# Autodesk Inventor assembly: Stage2
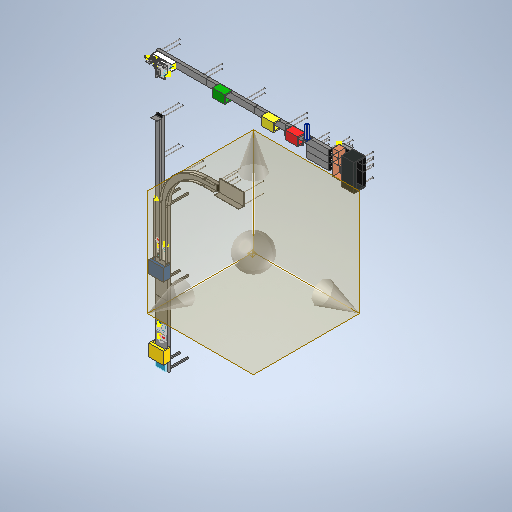
[picture p0: Inventor's stored thumbnail of the model, 512x512]
Saved by Autodesk Inventor 2025.1 (Build 291241000, 241)
## iProperties
Created: 2025-02-26
Part Number: Stage2
Document SubType Name: Assembly
Designer: yovan
Author: yovan
## Documents named in this file (27)
- C:\Users\yovan\Desktop\APM\ausol-apm.github.io\project\Design and simulation\Inventor\NXModeling\Stage2.iam
- C:\Users\yovan\Desktop\APM\ausol-apm.github.io\project\Design and simulation\Inventor\NXModeling\Assembler.ipt
- C:\Users\yovan\Desktop\APM\ausol-apm.github.io\project\Design and simulation\Inventor\NXModeling\ConveyorsStage2-3.ipt
- C:\Users\yovan\Desktop\APM\ausol-apm.github.io\project\Design and simulation\Inventor\Modelado juguetes\Barco\BarcoFinal.iam
- C:\Users\yovan\Desktop\APM\ausol-apm.github.io\project\Design and simulation\Inventor\Modelado juguetes\Barco\Piezabarcosuperior.ipt
- C:\Users\yovan\Desktop\APM\ausol-apm.github.io\project\Design and simulation\Inventor\Modelado juguetes\Barco\Timon.ipt
- C:\Users\yovan\Desktop\APM\ausol-apm.github.io\project\Design and simulation\Inventor\Modelado juguetes\Barco\PiezaTimon.ipt
- C:\Users\yovan\Desktop\APM\ausol-apm.github.io\project\Design and simulation\Inventor\Modelado juguetes\Moto\EnsamblajeMoto.iam
- C:\Users\yovan\Desktop\APM\ausol-apm.github.io\project\Design and simulation\Inventor\Modelado juguetes\Moto\Llanta.ipt
- C:\Users\yovan\Desktop\APM\ausol-apm.github.io\project\Design and simulation\Inventor\NXModeling\Sensor.ipt
- C:\Users\yovan\Desktop\APM\ausol-apm.github.io\project\Design and simulation\Inventor\Modelado juguetes\Casa\TechoCasa.ipt
- C:\Users\yovan\Desktop\APM\ausol-apm.github.io\project\Design and simulation\Inventor\Modelado juguetes\Casa\EnsamblajeCasa.iam
- C:\Users\yovan\Desktop\APM\ausol-apm.github.io\project\Design and simulation\Inventor\NXModeling\PneumaticActuator\PneummaticActuator.iam
- C:\Users\yovan\Desktop\APM\ausol-apm.github.io\project\Design and simulation\Inventor\NXModeling\Caja grande.ipt
- C:\Users\yovan\Desktop\APM\ausol-apm.github.io\project\Design and simulation\Inventor\NXModeling\Caja pequeña.ipt
- C:\Users\yovan\Desktop\APM\ausol-apm.github.io\project\Design and simulation\Inventor\NXModeling\ConveyorS&F.ipt
- C:\Users\yovan\Desktop\APM\ausol-apm.github.io\project\Design and simulation\Inventor\NXModeling\BiggerPneumatic\biggerAct.iam
- C:\Users\yovan\Desktop\APM\ausol-apm.github.io\project\Design and simulation\Inventor\NXModeling\Camera.ipt
- C:\Users\yovan\Desktop\APM\ausol-apm.github.io\project\Design and simulation\Inventor\NXModeling\smallerActuator\PneummaticActuatorSmall.iam
- C:\Users\yovan\Desktop\APM\ausol-apm.github.io\project\Design and simulation\Inventor\InjectionSetUp_RoboticCell\OutMold.ipt
- C:\Users\yovan\Desktop\APM\ausol-apm.github.io\project\Design and simulation\Inventor\Modelado juguetes\Casa\ParedDelanteraCasa.ipt
- C:\Users\yovan\Desktop\APM\ausol-apm.github.io\project\Design and simulation\Inventor\Modelado juguetes\Casa\ParedLateralCasa.ipt
- C:\Users\yovan\Desktop\APM\ausol-apm.github.io\project\Design and simulation\Inventor\Modelado juguetes\Casa\ParedTraseraCasa.ipt
- C:\Users\yovan\Desktop\APM\ausol-apm.github.io\project\Design and simulation\Inventor\Modelado juguetes\Casa\Puerta.ipt
- C:\Users\yovan\Desktop\APM\ausol-apm.github.io\project\Design and simulation\Inventor\Modelado juguetes\Casa\EnsamblajeCasaFinal.iam
- C:\Users\yovan\Desktop\APM\ausol-apm.github.io\project\Design and simulation\Inventor\Modelado juguetes\Moto\EnsamblajeMotoFinal.iam
- C:\Users\yovan\Desktop\APM\ausol-apm.github.io\project\Design and simulation\Inventor\Modelado juguetes\Barco\Inferior.ipt
## Components (71 placed, 26 different names)
1. Assembler:1 — Flush:1, Mate:1, Mate:3, Mate:4, Mate:8, Mate:9, Mate:10, Insert:4, Insert:5, Insert:6, Mate:11, Mate:12, Insert:7, Mate:13, Mate:14, Mate:15, Insert:8, Mate:16, Mate:17, Mate:18, Mate:19, Mate:20, Mate:21, Mate:24, Mate:25, Mate:26, Mate:27, Mate:28, Mate:29, Mate:30, Mate:39, Mate:40, Mate:42, Mate:43, Mate:83, Mate:84, Mate:85, Mate:86, Insert:9, Mate:89, Flush:37, Mate:90, Mate:91, Tangent:9, Tangent:10, Mate:94, Tangent:11
2. ConveyorsStage2-3:1 — Flush:1, Mate:1, Mate:31, Tangent:4, Flush:3, Tangent:5, Mate:32, Flush:4, Tangent:6, Mate:33, Flush:35, Tangent:7, Tangent:8, Flush:36, Mate:34, Mate:35, Mate:41, Mate:44, Mate:45, Mate:46, Mate:47, Mate:81, Mate:82
3. BarcoFinal:1 [sub-assembly] — Mate:89, Mate:91
4. Piezabarcosuperior:1 — Mate:3, Mate:4
5. Timon:1 — Mate:92, Mate:93, Flush:38
6. PiezaTimon:1 — Mate:92, Mate:93, Flush:38, Mate:94, Tangent:11
7. EnsamblajeMoto:1 [sub-assembly] — Mate:86
8. Llanta:1 — Mate:8, Tangent:9
9. Llanta:2 — Mate:9, Tangent:10
10. Sensor:1 — Insert:9
11. Sensor:2 — Mate:10
12. Sensor:3 — Mate:83
13. Sensor:4 — Insert:4
14. Sensor:5 — Insert:5
15. Sensor:6 — Insert:6
16. TechoCasa:1 — Mate:11, Mate:12
17. Sensor:7 — Insert:7
18. EnsamblajeCasa:1 [sub-assembly] — Mate:13, Mate:14, Mate:15
19. Sensor:8 — Insert:8
20. PneummaticActuator:1 [sub-assembly] — Mate:16, Mate:17
21. PneummaticActuator:2 [sub-assembly] — Mate:18, Mate:21
22. PneummaticActuator:3 [sub-assembly] — Mate:19, Mate:20
23. PneummaticActuator:4 [sub-assembly] — Mate:24, Mate:25
24. PneummaticActuator:5 [sub-assembly] — Mate:30
25. PneummaticActuator:6 [sub-assembly] — Mate:84, Mate:85
26. PneummaticActuator:7 [sub-assembly] — Mate:26
27. PneummaticActuator:9 [sub-assembly] — Mate:27, Mate:28
28. PneummaticActuator:10 [sub-assembly] — Mate:29
29. Caja grande:1 — Mate:31, Tangent:4, Flush:3
30. Caja pequeña:1 — Tangent:5, Mate:32, Flush:4
31. Caja pequeña:2 — Tangent:6, Mate:33, Flush:35
32. ConveyorS&F:1 — Tangent:7, Tangent:8, Flush:36, Mate:53, Mate:54, Mate:55, Mate:56, Mate:57, Mate:60, Mate:62, Mate:63, Mate:64, Mate:65, Mate:66, Mate:67, Mate:68, Mate:69, Mate:70, Mate:74, Mate:75, Mate:76, Mate:77, Mate:78, Mate:79, Mate:80, Mate:87, Mate:88
33. biggerAct:1 [sub-assembly] — Mate:34, Mate:35
34. Camera:1 — Mate:45, Mate:46, Mate:47
35. Sensor:9 — Mate:39
36. Sensor:10 — Mate:40
37. Sensor:11 — Mate:41
38. PneummaticActuatorSmall:1 [sub-assembly] — Mate:42, Mate:43
39. Sensor:12 — Mate:44
40. OutMold:2
41. ParedDelanteraCasa:1 — Mate:53
42. ParedLateralCasa:1 — Mate:55
43. ParedTraseraCasa:1 — Mate:54
44. Puerta:1 — Mate:57
45. TechoCasa:2 — Mate:56
46. Piezabarcosuperior:2 — Mate:60
47. Timon:2
48. PiezaTimon:2
49. EnsamblajeMoto:2 [sub-assembly] — Mate:62
50. Llanta:3 — Mate:63
51. Llanta:4 — Mate:64
52. Llanta:5 — Mate:65
53. Llanta:6 — Mate:66
54. ParedDelanteraCasa:2 — Mate:68
55. ParedLateralCasa:2 — Mate:67
56. ParedTraseraCasa:2 — Mate:69
57. Puerta:2 — Mate:70
58. TechoCasa:3 — Mate:80
59. Piezabarcosuperior:3 — Mate:74
60. Timon:3
61. PiezaTimon:3
62. EnsamblajeMoto:3 [sub-assembly] — Mate:75
63. Llanta:7 — Mate:77
64. Llanta:8 — Mate:79
65. Llanta:9 — Mate:78
66. Llanta:10 — Mate:76
67. EnsamblajeCasaFinal:1 [sub-assembly] — Mate:81
68. EnsamblajeMotoFinal:1 [sub-assembly] — Mate:82
69. Inferior:1 — Mate:87
70. Inferior:2 — Mate:88
71. Inferior:3 — Flush:37, Mate:90
## Relationships (95: Mate 74, Tangent 8, Flush 7, Insert 6)
- Flush:1 (-135 mm): Assembler:1 ↔ ConveyorsStage2-3:1
- Mate:1 (300 mm): Assembler:1 ↔ ConveyorsStage2-3:1
- Mate:3: Assembler:1 ↔ Piezabarcosuperior:1
- Mate:4: Assembler:1 ↔ Piezabarcosuperior:1
- Mate:8 (1.5 mm): Assembler:1 ↔ Llanta:1
- Mate:9 (1.5 mm): Assembler:1 ↔ Llanta:2
- Mate:10: Assembler:1 ↔ Sensor:2
- Insert:4 (-7 mm): Assembler:1 ↔ Sensor:4
- Insert:5 (-4 mm): Assembler:1 ↔ Sensor:5
- Insert:6 (-5 mm): Assembler:1 ↔ Sensor:6
- Mate:11: Assembler:1 ↔ TechoCasa:1
- Mate:12: Assembler:1 ↔ TechoCasa:1
- Insert:7 (-10 mm): Assembler:1 ↔ Sensor:7
- Mate:13: Assembler:1 ↔ EnsamblajeCasa:1
- Mate:14 (10 mm): Assembler:1 ↔ EnsamblajeCasa:1
- Mate:15: Assembler:1 ↔ EnsamblajeCasa:1
- Insert:8 (-7 mm): Assembler:1 ↔ Sensor:8
- Mate:16: Assembler:1 ↔ PneummaticActuator:1
- Mate:17 (10 mm): Assembler:1 ↔ PneummaticActuator:1
- Mate:18: Assembler:1 ↔ PneummaticActuator:2
- Mate:19: Assembler:1 ↔ PneummaticActuator:3
- Mate:20 (10 mm): Assembler:1 ↔ PneummaticActuator:3
- Mate:21 (10 mm): Assembler:1 ↔ PneummaticActuator:2
- Mate:24: Assembler:1 ↔ PneummaticActuator:4
- Mate:25 (10 mm): Assembler:1 ↔ PneummaticActuator:4
- Mate:26: Assembler:1 ↔ PneummaticActuator:7
- Mate:27: Assembler:1 ↔ PneummaticActuator:9
- Mate:28 (9 mm): Assembler:1 ↔ PneummaticActuator:9
- Mate:29: Assembler:1 ↔ PneummaticActuator:10
- Mate:30: Assembler:1 ↔ PneummaticActuator:5
- Mate:31: ConveyorsStage2-3:1 ↔ Caja grande:1
- Tangent:4 (-120 mm): ConveyorsStage2-3:1 ↔ Caja grande:1
- Flush:3: ConveyorsStage2-3:1 ↔ Caja grande:1
- Tangent:5 (-120 mm): ConveyorsStage2-3:1 ↔ Caja pequeña:1
- Mate:32: ConveyorsStage2-3:1 ↔ Caja pequeña:1
- Flush:4: ConveyorsStage2-3:1 ↔ Caja pequeña:1
- Tangent:6 (-120 mm): ConveyorsStage2-3:1 ↔ Caja pequeña:2
- Mate:33: ConveyorsStage2-3:1 ↔ Caja pequeña:2
- Flush:35: ConveyorsStage2-3:1 ↔ Caja pequeña:2
- Tangent:7 (2000 mm): ConveyorsStage2-3:1 ↔ ConveyorS&F:1
- Tangent:8 (-250 mm): ConveyorsStage2-3:1 ↔ ConveyorS&F:1
- Flush:36: ConveyorsStage2-3:1 ↔ ConveyorS&F:1
- Mate:34: ConveyorsStage2-3:1 ↔ biggerAct:1
- Mate:35: ConveyorsStage2-3:1 ↔ biggerAct:1
- Mate:39: Assembler:1 ↔ Sensor:9
- Mate:40: Assembler:1 ↔ Sensor:10
- Mate:41: ConveyorsStage2-3:1 ↔ Sensor:11
- Mate:42: Assembler:1 ↔ PneummaticActuatorSmall:1
- Mate:43 (15 mm): Assembler:1 ↔ PneummaticActuatorSmall:1
- Mate:44: ConveyorsStage2-3:1 ↔ Sensor:12
- Mate:45 (-20 mm): ConveyorsStage2-3:1 ↔ Camera:1
- Mate:46: ConveyorsStage2-3:1 ↔ Camera:1
- Mate:47: ConveyorsStage2-3:1 ↔ Camera:1
- Mate:53: ConveyorS&F:1 ↔ ParedDelanteraCasa:1
- Mate:54: ConveyorS&F:1 ↔ ParedTraseraCasa:1
- Mate:55: ConveyorS&F:1 ↔ ParedLateralCasa:1
- Mate:56: ConveyorS&F:1 ↔ TechoCasa:2
- Mate:57: ConveyorS&F:1 ↔ Puerta:1
- Mate:60: ConveyorS&F:1 ↔ Piezabarcosuperior:2
- Mate:62: ConveyorS&F:1 ↔ EnsamblajeMoto:2
- Mate:63: ConveyorS&F:1 ↔ Llanta:3
- Mate:64: ConveyorS&F:1 ↔ Llanta:4
- Mate:65: ConveyorS&F:1 ↔ Llanta:5
- Mate:66: ConveyorS&F:1 ↔ Llanta:6
- Mate:67: ConveyorS&F:1 ↔ ParedLateralCasa:2
- Mate:68: ConveyorS&F:1 ↔ ParedDelanteraCasa:2
- Mate:69: ConveyorS&F:1 ↔ ParedTraseraCasa:2
- Mate:70: ConveyorS&F:1 ↔ Puerta:2
- Mate:74: ConveyorS&F:1 ↔ Piezabarcosuperior:3
- Mate:75: ConveyorS&F:1 ↔ EnsamblajeMoto:3
- Mate:76: ConveyorS&F:1 ↔ Llanta:10
- Mate:77: ConveyorS&F:1 ↔ Llanta:7
- Mate:78: ConveyorS&F:1 ↔ Llanta:9
- Mate:79: ConveyorS&F:1 ↔ Llanta:8
- Mate:80: ConveyorS&F:1 ↔ TechoCasa:3
- Mate:81 (100 mm): ConveyorsStage2-3:1 ↔ EnsamblajeCasaFinal:1
- Mate:82 (230 mm): ConveyorsStage2-3:1 ↔ EnsamblajeMotoFinal:1
- Mate:83: Assembler:1 ↔ Sensor:3
- Mate:84: Assembler:1 ↔ PneummaticActuator:6
- Mate:85 (15 mm): Assembler:1 ↔ PneummaticActuator:6
- Mate:86: Assembler:1 ↔ EnsamblajeMoto:1
- Insert:9 (2 mm): Assembler:1 ↔ Sensor:1
- Mate:87: ConveyorS&F:1 ↔ Inferior:1
- Mate:88: ConveyorS&F:1 ↔ Inferior:2
- Mate:89 (10 mm): Assembler:1 ↔ BarcoFinal:1
- Flush:37 (-25 mm): Assembler:1 ↔ Inferior:3
- Mate:90: Assembler:1 ↔ Inferior:3
- Mate:91: Assembler:1 ↔ BarcoFinal:1
- Tangent:9 (1 mm): Assembler:1 ↔ Llanta:1
- Tangent:10 (2 mm): Assembler:1 ↔ Llanta:2
- Mate:92: Timon:1 ↔ PiezaTimon:1
- Mate:93: Timon:1 ↔ PiezaTimon:1
- Flush:38: Timon:1 ↔ PiezaTimon:1
- Mate:94: Assembler:1 ↔ PiezaTimon:1
- Tangent:11: Assembler:1 ↔ PiezaTimon:1
